# Autodesk Inventor assembly: Assembly Mount Base
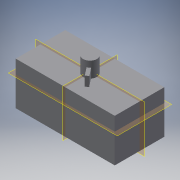
[picture p0: Inventor's stored thumbnail of the model, 180x180]
Saved by Autodesk Inventor 2019 (Build 230136000, 136)
## iProperties
Created: 2021-05-14
Part Number: Assembly Mount Base
Document SubType Name: Assembly
Designer: Eric
Author: Eric
## Documents named in this file (4)
- C:\Users\Eric\Documents\! - Uni\Year 4\MENG-Robot-Fab-Project\Models\For_Optimiser\Static Parts Assembly\Assembly Mount Assembly\Assembly Mount Base.iam
- C:\Users\Eric\Documents\! - Uni\Year 4\MENG-Robot-Fab-Project\Models\For_Optimiser\Static Parts Assembly\Assembly Mount Assembly\AssemblyMountBase_body.ipt
- C:\Users\Eric\Documents\! - Uni\Year 4\MENG-Robot-Fab-Project\Models\For_Optimiser\Static Parts Assembly\Assembly Mount Assembly\AssemblyMountBase_axle.ipt
- C:\Users\Eric\Documents\! - Uni\Year 4\MENG-Robot-Fab-Project\Models\For_Optimiser\Static Parts Assembly\Assembly Mount Assembly\AssemblyMountBase_sensor.ipt
## Components (3 placed, 3 different names)
1. AssemblyMountBase_body:1 — Symmetry:1
2. AssemblyMountBase_axle:1 — Symmetry:1
3. AssemblyMountBase_sensor:1
## Relationships (1: Symmetry 1)
- Symmetry:1: AssemblyMountBase_body:1 ↔ AssemblyMountBase_axle:1
